# Autodesk Inventor assembly: ImpresionBordes
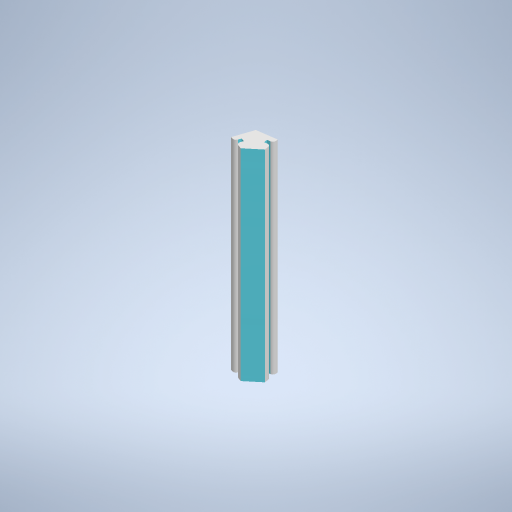
[picture p0: Inventor's stored thumbnail of the model, 512x512]
Saved by Autodesk Inventor 2024 (Build 280153000, 153)
## iProperties
Created: 2024-04-21
Part Number: ImpresionBordes
Document SubType Name: Assembly
Designer: sergi
Author: sergi
## Documents named in this file (3)
- C:\Users\sergi\OneDrive\Escritorio\proyectos\Piso\Dodecaedro\ImpresionBordes.iam
- C:\Users\sergi\OneDrive\Escritorio\proyectos\Piso\Dodecaedro\Perfil_V3.ipt
- C:\Users\sergi\OneDrive\Escritorio\proyectos\Piso\Dodecaedro\auxiliar.ipt
## Components (2 placed, 2 different names)
1. Perfil_V3:1 — Coincidencia:1, Ángulo:1
2. auxiliar:1 — Coincidencia:1, Ángulo:1
## Relationships (2: Mate 1, Angle 1)
- Coincidencia:1 [Mate]: Perfil_V3:1 ↔ auxiliar:1
- Ángulo:1 [Angle] (108.435 deg): Perfil_V3:1 ↔ auxiliar:1
